# Autodesk Inventor assembly: Assembly_Cube_Flashlight_v3
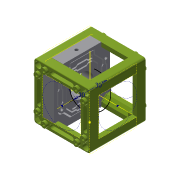
[picture p0: Inventor's stored thumbnail of the model, 180x180]
Saved by Autodesk Inventor 2019.4 (Build 234330000, 330)
## iProperties
Created: 2020-12-04
Part Number: Assembly_Cube_Flashlight_v3
Document SubType Name: Assembly
Designer: UC2
Author: UC2
## Documents named in this file (3)
- C:\Users\diederichbenedict\Dropbox\Dokumente\Promotion\PROJECTS\UC2\02_CAD\INVENTOR\uc2_v3\Assembly_Cube_Flexuremanipulator_v3.iam
- C:\Users\diederichbenedict\Dropbox\Dokumente\Promotion\PROJECTS\UC2\02_CAD\INVENTOR\uc2_v3\Assembly_Cube_empty_IM_v3.iam
- C:\Users\diederichbenedict\Dropbox\Dokumente\Promotion\PROJECTS\UC2\02_CAD\INVENTOR\uc2_v3\20_Cube_Inser_Flexuremanipulator_v3.ipt
## Components (2 placed, 2 different names)
1. Assembly_Cube_empty_IM_v3:1 [sub-assembly] — Flush:3, Flush:4
2. 20_Cube_Inser_Flexuremanipulator_v3:1 — Flush:3, Flush:4
## Relationships (2: Flush 2)
- Flush:3: Assembly_Cube_empty_IM_v3:1 ↔ 20_Cube_Inser_Flexuremanipulator_v3:1
- Flush:4: Assembly_Cube_empty_IM_v3:1 ↔ 20_Cube_Inser_Flexuremanipulator_v3:1
